# Autodesk Inventor assembly: Assembly Bumper
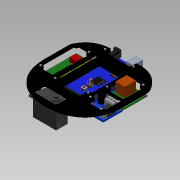
[picture p0: Inventor's stored thumbnail of the model, 180x180]
Saved by Autodesk Inventor 2015 SP1 (Build 190203100, 203)
## iProperties
Created: 2015-02-05
Part Number: Assembly Bumper
Document SubType Name: Assembly
Designer: Rafi Kurnia Putra
Author: Rafi Kurnia Putra
## Documents named in this file (8)
- D:\Dropbox\krpai berkaki trui 2015\ROBUSTA\MEKANIK\ROBUSTA\Assembly Bumper.iam
- D:\Dropbox\krpai berkaki trui 2015\ROBUSTA\MEKANIK\ROBUSTA\bumper.ipt
- D:\Dropbox\krpai berkaki trui 2015\ROBUSTA\MEKANIK\ROBUSTA\DC to DC Converter.ipt
- D:\Dropbox\krpai berkaki trui 2015\ROBUSTA\MEKANIK\ROBUSTA\Driver Kipas v2.ipt
- D:\Dropbox\krpai berkaki trui 2015\ROBUSTA\MEKANIK\ROBUSTA\Spacer 1cm.ipt
- D:\Dropbox\krpai berkaki trui 2015\ROBUSTA\MEKANIK\ROBUSTA\Arduino Mega.ipt
- D:\Dropbox\krpai berkaki trui 2015\ROBUSTA\MEKANIK\ROBUSTA\Mode V2.ipt
- D:\Dropbox\krpai berkaki trui 2015\ROBUSTA\MEKANIK\ROBUSTA\servo.ipt
## Components (15 placed, 7 different names)
1. bumper:1 — Mate:1, Mate:2, Mate:3, Mate:4, Mate:7, Mate:8, Angle:1, Mate:15, Mate:16, Mate:17, Mate:30, Mate:31, Mate:32, Angle:3, Mate:33, Mate:34, Mate:36, Mate:37, Mate:44, Mate:45
2. servo:1 — Mate:4, Mate:44, Mate:45
3. Spacer 1cm:1 — Mate:7, Mate:8, Mate:9, Mate:10
4. Spacer 1cm:4 — Mate:14, Mate:15, Mate:17, Mate:46
5. Spacer 1cm:5 — Mate:13, Mate:16, Mate:47
6. Spacer 1cm:6 — Mate:23, Mate:26, Mate:31
7. Spacer 1cm:7 — Mate:25, Mate:29, Mate:32
8. Spacer 1cm:8 — Mate:24, Mate:28, Mate:30
9. Spacer 1cm:9 — Mate:22, Mate:27
10. DC to DC Converter:1 — Mate:9, Mate:10, Angle:1
11. Driver Kipas v2:1 — Mate:13, Mate:14, Mate:46, Mate:47
12. Arduino Mega:1 — Mate:22, Mate:23, Mate:24, Mate:25, Mate:26, Mate:27, Mate:28, Mate:29
13. Mode V2:1 — Angle:3, Mate:35, Mate:48
14. Spacer 1cm:11 — Mate:33, Mate:34, Mate:35
15. Spacer 1cm:10 — Mate:36, Mate:37, Mate:48
## Relationships (36: Mate 34, Angle 2)
- Mate:1: bumper:1
- Mate:2: bumper:1
- Mate:3: bumper:1
- Mate:4 (5 mm): bumper:1 ↔ servo:1
- Mate:7: bumper:1 ↔ Spacer 1cm:1
- Mate:8: bumper:1 ↔ Spacer 1cm:1
- Mate:9: Spacer 1cm:1 ↔ DC to DC Converter:1
- Mate:10: Spacer 1cm:1 ↔ DC to DC Converter:1
- Angle:1 (0 deg): bumper:1 ↔ DC to DC Converter:1
- Mate:13: Spacer 1cm:5 ↔ Driver Kipas v2:1
- Mate:14: Spacer 1cm:4 ↔ Driver Kipas v2:1
- Mate:15: bumper:1 ↔ Spacer 1cm:4
- Mate:16: bumper:1 ↔ Spacer 1cm:5
- Mate:17: bumper:1 ↔ Spacer 1cm:4
- Mate:22: Spacer 1cm:9 ↔ Arduino Mega:1
- Mate:23: Spacer 1cm:6 ↔ Arduino Mega:1
- Mate:24: Spacer 1cm:8 ↔ Arduino Mega:1
- Mate:25: Spacer 1cm:7 ↔ Arduino Mega:1
- Mate:26: Spacer 1cm:6 ↔ Arduino Mega:1
- Mate:27: Spacer 1cm:9 ↔ Arduino Mega:1
- Mate:28: Spacer 1cm:8 ↔ Arduino Mega:1
- Mate:29: Spacer 1cm:7 ↔ Arduino Mega:1
- Mate:30: bumper:1 ↔ Spacer 1cm:8
- Mate:31: bumper:1 ↔ Spacer 1cm:6
- Mate:32: bumper:1 ↔ Spacer 1cm:7
- Angle:3 (0 deg): bumper:1 ↔ Mode V2:1
- Mate:33: bumper:1 ↔ Spacer 1cm:11
- Mate:34: bumper:1 ↔ Spacer 1cm:11
- Mate:35: Mode V2:1 ↔ Spacer 1cm:11
- Mate:36: bumper:1 ↔ Spacer 1cm:10
- Mate:37: bumper:1 ↔ Spacer 1cm:10
- Mate:44: bumper:1 ↔ servo:1
- Mate:45: bumper:1 ↔ servo:1
- Mate:46: Spacer 1cm:4 ↔ Driver Kipas v2:1
- Mate:47: Spacer 1cm:5 ↔ Driver Kipas v2:1
- Mate:48: Mode V2:1 ↔ Spacer 1cm:10
